# Autodesk Inventor assembly: dtmotorgearsdeadaxle_MIR1
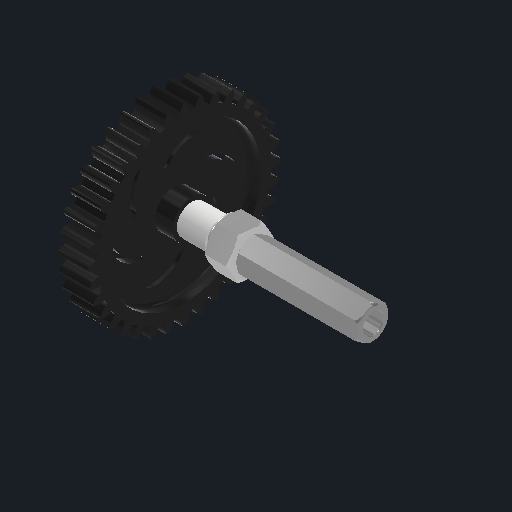
[picture p0: Inventor's stored thumbnail of the model, 512x512]
Saved by Autodesk Inventor 2026.1 (Build 301233000, 233)
## iProperties
Created: 2025-08-03
Part Number: dtmotorgearsdeadaxle_MIR1
Document SubType Name: Assembly
Designer: roejo
Author: roejo
## Documents named in this file (8)
- C:\Users\roejo\OneDrive\Documents\2026WorldChampionRobot\Robots\Worlds\Subassemblies\dtmotorgearsdeadaxle_MIR1.iam
- C:\Users\roejo\OneDrive\Documents\2026WorldChampionRobot\Library\VEX-CAD-Inventor-1.4.2\Motion\Gears\LS 36T Gear_MIR1.ipt
- C:\Users\roejo\OneDrive\Documents\2026WorldChampionRobot\Library\VEX-CAD-Inventor-1.4.2\Motion\Spacers\Washer Teflon\TWasher .375 OD x .06250.ipt
- C:\Users\roejo\OneDrive\Documents\2026WorldChampionRobot\Library\VEX-CAD-Inventor-1.4.2\Motion\Spacers\Washer Teflon.ipt
- C:\Users\roejo\OneDrive\Documents\2026WorldChampionRobot\Library\VEX-CAD-Inventor-1.4.2\Structure\Hardware\alu_nylock_MIR1.ipt
- C:\Users\roejo\OneDrive\Documents\2026WorldChampionRobot\Library\VEX-CAD-Inventor-1.4.2\Structure\Standoff\Standoff 1.00.ipt
- C:\Users\roejo\OneDrive\Documents\2026WorldChampionRobot\Library\VEX-CAD-Inventor-1.4.2\Structure\Standoff.ipt
- C:\Users\roejo\OneDrive\Documents\2026WorldChampionRobot\Library\VEX-CAD-Inventor-1.4.2\Motion\Spacers\thinspacer0.25_MIR2.ipt
## Components (5 placed, 5 different names)
1. LS 36T Gear_MIR1:1 — Insert:1, Insert:4
2. TWasher .375 OD x .06250:1 — Insert:1
3. alu_nylock_MIR1:1 — Insert:2, Insert:3
4. Standoff 1.00:1 — Insert:2
5. thinspacer0.25_MIR2:1 — Insert:4, Insert:3
## Relationships (4: Insert 4)
- Insert:1: LS 36T Gear_MIR1:1 ↔ TWasher .375 OD x .06250:1
- Insert:2: alu_nylock_MIR1:1 ↔ Standoff 1.00:1
- Insert:4: LS 36T Gear_MIR1:1 ↔ thinspacer0.25_MIR2:1
- Insert:3: alu_nylock_MIR1:1 ↔ thinspacer0.25_MIR2:1
